# Autodesk Inventor assembly: assembly_cnv
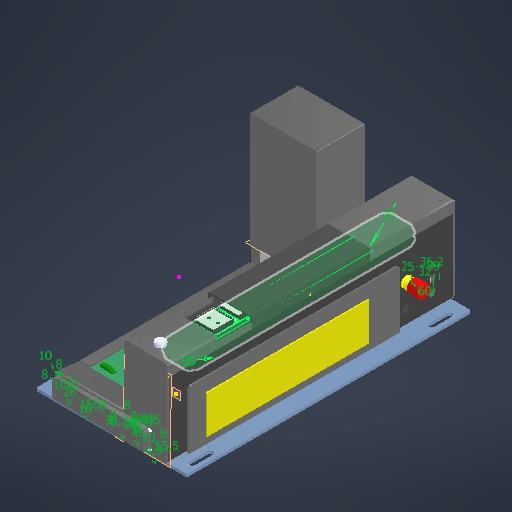
[picture p0: Inventor's stored thumbnail of the model, 512x512]
Saved by Autodesk Inventor 2026.1 (Build 301233020, 233B)
## iProperties
Created: 2025-08-17
Part Number: assembly_cnv
Document SubType Name: Assembly
Designer: peter
Author: peter
## Documents named in this file (3)
- C:\Users\neume\Desktop\MCI\Robotik_Projekt\Optimierung-Laboraufgabe-Robotik\Abgabe_Optimierung_Robotik\Konstruktion\Inventor_ConveyorTracking\assembly_cnv.iam
- C:\Users\neume\Desktop\MCI\Robotik_Projekt\Optimierung-Laboraufgabe-Robotik\Abgabe_Optimierung_Robotik\Konstruktion\Inventor_ConveyorTracking\FakeMachineV2.iam
- C:\Users\neume\Desktop\MCI\Robotik_Projekt\Optimierung-Laboraufgabe-Robotik\Abgabe_Optimierung_Robotik\Konstruktion\Inventor_ConveyorTracking\Bildverarbeitungsband_Blech.iam
## Components (2 placed, 2 different names)
1. FakeMachineV2:1 [sub-assembly] — Fluchtend:1
2. Bildverarbeitungsband_Blech:1 [sub-assembly] — Fluchtend:1
## Relationships (1: Flush 1)
- Fluchtend:1 [Flush]: FakeMachineV2:1 ↔ Bildverarbeitungsband_Blech:1
